# Autodesk Inventor assembly: Backhoe
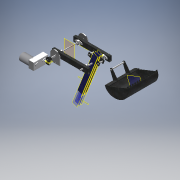
[picture p0: Inventor's stored thumbnail of the model, 180x180]
Saved by Autodesk Inventor 2019 (Build 230136000, 136)
## iProperties
Created: 2018-10-28
Part Number: Backhoe
Document SubType Name: Assembly
Designer: Alex Barnett
Author: Alex Barnett
## Documents named in this file (16)
- C:\Users\Alex Barnett\Documents\Machine Design\PR2\CAD\Backhoe.iam
- C:\Users\Alex Barnett\Documents\Machine Design\PR2\CAD\Boom Hinge.ipt
- C:\Users\Alex Barnett\Documents\Machine Design\PR2\CAD\Pin .5in. Dia. - Boom Hinge.ipt
- C:\Users\Alex Barnett\Documents\Machine Design\PR2\CAD\Ball Bearing .5in..ipt
- C:\Users\Alex Barnett\Documents\Machine Design\PR2\CAD\Steel 4130 1x2in. Tubing, t=.065in.,L=15in..ipt
- C:\Users\Alex Barnett\Documents\Machine Design\PR2\CAD\Steel 4130 1x2in. Tubing, t=.065in.,L=22in..ipt
- C:\Users\Alex Barnett\Documents\Machine Design\PR2\CAD\Flange-Mount Sealed Ball Bearing .5in. Dia..ipt
- C:\Users\Alex Barnett\Documents\Machine Design\PR2\CAD\Boom to Stick .5in. Pin.ipt
- C:\Users\Alex Barnett\Documents\Machine Design\PR2\CAD\AmpFlow Motor & Gearbox.iam
- C:\Users\Alex Barnett\Documents\Machine Design\PR2\CAD\Worm Gear 12P 18T.ipt
- C:\Users\Alex Barnett\Documents\Machine Design\PR2\CAD\Steel 4130 1x2in. Tubing, t=.065in.,L=22in. Mirrored.ipt
- C:\Users\Alex Barnett\Documents\Machine Design\PR2\CAD\Stick to Scoop .5in. Pin.ipt
- C:\Users\Alex Barnett\Documents\Machine Design\PR2\CAD\Bucket.ipt
- C:\Users\Alex Barnett\Documents\Machine Design\PR2\CAD\Linear Actuator Top Pin .5in. Dia..ipt
- C:\Users\Alex Barnett\Documents\Machine Design\PR2\CAD\Linear Actuator Top Scoop Pin .5in. Dia..ipt
- C:\Users\Alex Barnett\Documents\Machine Design\PR2\CAD\Dry-Running Two-Bolt Flange Mounted Bearing, 0.5in. Diameter.ipt
## Components (25 placed, 15 different names)
1. Boom Hinge:1 — Mate:1, Mate:2, Mate:3, Flush:2, Mate:6, Mate:7, Flush:3, Mate:14, Flush:24
2. Boom Hinge:2 — Mate:5, Flush:2, Mate:8, Flush:4, Flush:5, Mate:14, Mate:54, Flush:11
3. Pin .5in. Dia. - Boom Hinge:1 — Mate:5, Mate:6, Flush:5, Mate:21, Mate:54, Mate:67, Mate:68, Flush:16, Flush:23, Mate:105, Mate:108
4. Ball Bearing .5in.:1 — Mate:7, Flush:3
5. Ball Bearing .5in.:2 — Mate:8, Flush:4
6. Steel 4130 1x2in. Tubing, t=.065in.,L=15in.:1 — Flush:6, Mate:21, Mate:32, Mate:33, Mate:34, Flush:23, Mate:104, Mate:106, Mate:110, Mate:112, Mate:113
7. Steel 4130 1x2in. Tubing, t=.065in.,L=15in.:2 — Flush:6, Mate:29, Mate:30, Mate:31, Mate:107, Mate:109, Mate:114, Mate:116
8. Flange-Mount Sealed Ball Bearing .5in. Dia.:1 — Mate:29, Mate:30, Mate:31, Mate:35, Flush:8
9. Flange-Mount Sealed Ball Bearing .5in. Dia.:2 — Mate:32, Mate:33, Mate:34
10. Boom to Stick .5in. Pin:1 — Mate:35, Flush:8, Mate:72, Mate:73, Mate:80, Mate:111, Mate:113, Mate:115
11. AmpFlow Motor & Gearbox:1 [sub-assembly] — Mate:69, Mate:70, Mate:71
12. Worm Gear 12P 18T:1 — Mate:67, Mate:68, Flush:16, Mate:69, Mate:70, Mate:71
13. Steel 4130 1x2in. Tubing, t=.065in.,L=22in.:1 — Mate:72, Mate:73, Mate:77, Mate:78, Mate:79, Flush:17, Mate:84, Flush:19, Mate:95
14. Flange-Mount Sealed Ball Bearing .5in. Dia.:3 — Mate:77, Mate:78, Mate:79
15. Steel 4130 1x2in. Tubing, t=.065in.,L=22in. Mirrored:1 — Mate:80, Flush:17, Mate:84, Mate:85, Mate:86, Mate:87, Flush:18, Mate:91, Flush:21, Flush:22, Mate:103
16. Flange-Mount Sealed Ball Bearing .5in. Dia.:4 — Mate:85, Mate:86, Mate:87, Mate:88
17. Stick to Scoop .5in. Pin:1 — Mate:88, Flush:18, Mate:89
18. Bucket:1 — Mate:89, Flush:19, Mate:93, Mate:94
19. Linear Actuator Top Pin .5in. Dia.:1 — Mate:91, Flush:21
20. Linear Actuator Top Scoop Pin .5in. Dia.:1 — Mate:93, Mate:94
21. Linear Actuator Top Pin .5in. Dia.:2 — Mate:95, Flush:22
22. Dry-Running Two-Bolt Flange Mounted Bearing, 0.5in. Diameter:3 — Mate:104, Mate:105, Mate:106
23. Dry-Running Two-Bolt Flange Mounted Bearing, 0.5in. Diameter:4 — Mate:107, Mate:108, Mate:109
24. Dry-Running Two-Bolt Flange Mounted Bearing, 0.5in. Diameter:5 — Mate:110, Mate:111, Mate:112
25. Dry-Running Two-Bolt Flange Mounted Bearing, 0.5in. Diameter:6 — Mate:114, Mate:115, Mate:116
## Relationships (69: Mate 52, Flush 17)
- Mate:1: Boom Hinge:1
- Mate:2: Boom Hinge:1
- Mate:3: Boom Hinge:1
- Mate:5: Boom Hinge:2 ↔ Pin .5in. Dia. - Boom Hinge:1
- Flush:2: Boom Hinge:1 ↔ Boom Hinge:2
- Mate:6: Boom Hinge:1 ↔ Pin .5in. Dia. - Boom Hinge:1
- Mate:7: Boom Hinge:1 ↔ Ball Bearing .5in.:1
- Flush:3: Boom Hinge:1 ↔ Ball Bearing .5in.:1
- Mate:8: Boom Hinge:2 ↔ Ball Bearing .5in.:2
- Flush:4: Boom Hinge:2 ↔ Ball Bearing .5in.:2
- Flush:5: Boom Hinge:2 ↔ Pin .5in. Dia. - Boom Hinge:1
- Mate:14 (-304.8 mm): Boom Hinge:1 ↔ Boom Hinge:2
- Flush:6: Steel 4130 1x2in. Tubing, t=.065in.,L=15in.:1 ↔ Steel 4130 1x2in. Tubing, t=.065in.,L=15in.:2
- Mate:21: Pin .5in. Dia. - Boom Hinge:1 ↔ Steel 4130 1x2in. Tubing, t=.065in.,L=15in.:1
- Mate:29: Steel 4130 1x2in. Tubing, t=.065in.,L=15in.:2 ↔ Flange-Mount Sealed Ball Bearing .5in. Dia.:1
- Mate:30: Steel 4130 1x2in. Tubing, t=.065in.,L=15in.:2 ↔ Flange-Mount Sealed Ball Bearing .5in. Dia.:1
- Mate:31: Steel 4130 1x2in. Tubing, t=.065in.,L=15in.:2 ↔ Flange-Mount Sealed Ball Bearing .5in. Dia.:1
- Mate:32: Steel 4130 1x2in. Tubing, t=.065in.,L=15in.:1 ↔ Flange-Mount Sealed Ball Bearing .5in. Dia.:2
- Mate:33: Steel 4130 1x2in. Tubing, t=.065in.,L=15in.:1 ↔ Flange-Mount Sealed Ball Bearing .5in. Dia.:2
- Mate:34: Steel 4130 1x2in. Tubing, t=.065in.,L=15in.:1 ↔ Flange-Mount Sealed Ball Bearing .5in. Dia.:2
- Mate:35: Flange-Mount Sealed Ball Bearing .5in. Dia.:1 ↔ Boom to Stick .5in. Pin:1
- Flush:8: Flange-Mount Sealed Ball Bearing .5in. Dia.:1 ↔ Boom to Stick .5in. Pin:1
- Mate:54: Boom Hinge:2 ↔ Pin .5in. Dia. - Boom Hinge:1
- Flush:11: Boom Hinge:2
- Flush:12 (300 mm)
- Flush:13 (500 mm)
- Mate:67: Pin .5in. Dia. - Boom Hinge:1 ↔ Worm Gear 12P 18T:1
- Mate:68: Pin .5in. Dia. - Boom Hinge:1 ↔ Worm Gear 12P 18T:1
- Flush:16: Pin .5in. Dia. - Boom Hinge:1 ↔ Worm Gear 12P 18T:1
- Mate:69: AmpFlow Motor & Gearbox:1 ↔ Worm Gear 12P 18T:1
- Mate:70: AmpFlow Motor & Gearbox:1 ↔ Worm Gear 12P 18T:1
- Mate:71: AmpFlow Motor & Gearbox:1 ↔ Worm Gear 12P 18T:1
- Mate:72: Boom to Stick .5in. Pin:1 ↔ Steel 4130 1x2in. Tubing, t=.065in.,L=22in.:1
- Mate:73: Boom to Stick .5in. Pin:1 ↔ Steel 4130 1x2in. Tubing, t=.065in.,L=22in.:1
- Mate:77: Steel 4130 1x2in. Tubing, t=.065in.,L=22in.:1 ↔ Flange-Mount Sealed Ball Bearing .5in. Dia.:3
- Mate:78: Steel 4130 1x2in. Tubing, t=.065in.,L=22in.:1 ↔ Flange-Mount Sealed Ball Bearing .5in. Dia.:3
- Mate:79: Steel 4130 1x2in. Tubing, t=.065in.,L=22in.:1 ↔ Flange-Mount Sealed Ball Bearing .5in. Dia.:3
- Mate:80: Boom to Stick .5in. Pin:1 ↔ Steel 4130 1x2in. Tubing, t=.065in.,L=22in. Mirrored:1
- Flush:17: Steel 4130 1x2in. Tubing, t=.065in.,L=22in.:1 ↔ Steel 4130 1x2in. Tubing, t=.065in.,L=22in. Mirrored:1
- Mate:84: Steel 4130 1x2in. Tubing, t=.065in.,L=22in.:1 ↔ Steel 4130 1x2in. Tubing, t=.065in.,L=22in. Mirrored:1
- Mate:85: Steel 4130 1x2in. Tubing, t=.065in.,L=22in. Mirrored:1 ↔ Flange-Mount Sealed Ball Bearing .5in. Dia.:4
- Mate:86: Steel 4130 1x2in. Tubing, t=.065in.,L=22in. Mirrored:1 ↔ Flange-Mount Sealed Ball Bearing .5in. Dia.:4
- Mate:87: Steel 4130 1x2in. Tubing, t=.065in.,L=22in. Mirrored:1 ↔ Flange-Mount Sealed Ball Bearing .5in. Dia.:4
- Mate:88: Flange-Mount Sealed Ball Bearing .5in. Dia.:4 ↔ Stick to Scoop .5in. Pin:1
- Flush:18: Steel 4130 1x2in. Tubing, t=.065in.,L=22in. Mirrored:1 ↔ Stick to Scoop .5in. Pin:1
- Mate:89: Stick to Scoop .5in. Pin:1 ↔ Bucket:1
- Flush:19: Steel 4130 1x2in. Tubing, t=.065in.,L=22in.:1 ↔ Bucket:1
- Mate:91: Steel 4130 1x2in. Tubing, t=.065in.,L=22in. Mirrored:1 ↔ Linear Actuator Top Pin .5in. Dia.:1
- Flush:21: Steel 4130 1x2in. Tubing, t=.065in.,L=22in. Mirrored:1 ↔ Linear Actuator Top Pin .5in. Dia.:1
- Mate:93: Bucket:1 ↔ Linear Actuator Top Scoop Pin .5in. Dia.:1
- Mate:94: Bucket:1 ↔ Linear Actuator Top Scoop Pin .5in. Dia.:1
- Mate:95: Steel 4130 1x2in. Tubing, t=.065in.,L=22in.:1 ↔ Linear Actuator Top Pin .5in. Dia.:2
- Flush:22: Steel 4130 1x2in. Tubing, t=.065in.,L=22in. Mirrored:1 ↔ Linear Actuator Top Pin .5in. Dia.:2
- Flush:23: Pin .5in. Dia. - Boom Hinge:1 ↔ Steel 4130 1x2in. Tubing, t=.065in.,L=15in.:1
- Flush:24 (-152.4 mm): Boom Hinge:1
- Mate:103: Steel 4130 1x2in. Tubing, t=.065in.,L=22in. Mirrored:1
- Mate:104: Steel 4130 1x2in. Tubing, t=.065in.,L=15in.:1 ↔ Dry-Running Two-Bolt Flange Mounted Bearing, 0.5in. Diameter:3
- Mate:105: Pin .5in. Dia. - Boom Hinge:1 ↔ Dry-Running Two-Bolt Flange Mounted Bearing, 0.5in. Diameter:3
- Mate:106: Steel 4130 1x2in. Tubing, t=.065in.,L=15in.:1 ↔ Dry-Running Two-Bolt Flange Mounted Bearing, 0.5in. Diameter:3
- Mate:107: Steel 4130 1x2in. Tubing, t=.065in.,L=15in.:2 ↔ Dry-Running Two-Bolt Flange Mounted Bearing, 0.5in. Diameter:4
- Mate:108: Pin .5in. Dia. - Boom Hinge:1 ↔ Dry-Running Two-Bolt Flange Mounted Bearing, 0.5in. Diameter:4
- Mate:109: Steel 4130 1x2in. Tubing, t=.065in.,L=15in.:2 ↔ Dry-Running Two-Bolt Flange Mounted Bearing, 0.5in. Diameter:4
- Mate:110: Steel 4130 1x2in. Tubing, t=.065in.,L=15in.:1 ↔ Dry-Running Two-Bolt Flange Mounted Bearing, 0.5in. Diameter:5
- Mate:111: Boom to Stick .5in. Pin:1 ↔ Dry-Running Two-Bolt Flange Mounted Bearing, 0.5in. Diameter:5
- Mate:112: Steel 4130 1x2in. Tubing, t=.065in.,L=15in.:1 ↔ Dry-Running Two-Bolt Flange Mounted Bearing, 0.5in. Diameter:5
- Mate:113: Steel 4130 1x2in. Tubing, t=.065in.,L=15in.:1 ↔ Boom to Stick .5in. Pin:1
- Mate:114: Steel 4130 1x2in. Tubing, t=.065in.,L=15in.:2 ↔ Dry-Running Two-Bolt Flange Mounted Bearing, 0.5in. Diameter:6
- Mate:115: Boom to Stick .5in. Pin:1 ↔ Dry-Running Two-Bolt Flange Mounted Bearing, 0.5in. Diameter:6
- Mate:116: Steel 4130 1x2in. Tubing, t=.065in.,L=15in.:2 ↔ Dry-Running Two-Bolt Flange Mounted Bearing, 0.5in. Diameter:6
